# Autodesk Inventor assembly: Pulley assembly
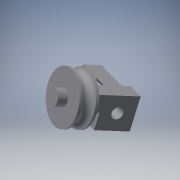
[picture p0: Inventor's stored thumbnail of the model, 180x180]
Saved by Autodesk Inventor 2019 (Build 230136000, 136)
## iProperties
Created: 2019-05-30
Part Number: Pulley assembly
Document SubType Name: Assembly
Designer: Delta
Author: Delta
## Documents named in this file (4)
- C:\Robotics\2019-20_CAD\Linear Slides\Pulley assembly.iam
- C:\Robotics\2019-20_CAD\offseason\random ideas\end peice for slides left.ipt
- C:\Robotics\2018-19_CAD\3d printer\pulley alpha.ipt
- C:\Robotics\2019-20_CAD\Linear Slides\screw for pulley.ipt
## Components (3 placed, 3 different names)
1. end peice for slides left:1 — Mate:1, Mate:2, Mate:5
2. pulley alpha:1 — Mate:1, Mate:2, Mate:4
3. screw for pulley:1 — Mate:4, Mate:5
## Relationships (4: Mate 4)
- Mate:1: end peice for slides left:1 ↔ pulley alpha:1
- Mate:2: end peice for slides left:1 ↔ pulley alpha:1
- Mate:4: pulley alpha:1 ↔ screw for pulley:1
- Mate:5: end peice for slides left:1 ↔ screw for pulley:1
